# Autodesk Inventor assembly: 00A-200 2019 GreyT Claw
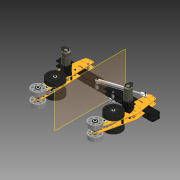
[picture p0: Inventor's stored thumbnail of the model, 180x180]
Saved by Autodesk Inventor 2022 (Build 260153000, 153)
## iProperties
RuleStatus: InUse
Created: 2020-10-29
Part Number: 00A-200 2019 GreyT Claw
Document SubType Name: Assembly
## Documents named in this file (44)
- C:\Users\Cal\Desktop\Robotics\Design\Collaborative\Collaborative Parts Library\Standard Order Parts\GreyT Claw Configurations\GreyT Claw.iam
- C:\Users\Cal\Desktop\Robotics\Design\Collaborative\Collaborative Parts Library\Standard Order Parts\GreyT Claw Configurations\GreyT Claw Top V2.ipt
- C:\Users\Cal\Desktop\Robotics\Design\Collaborative\Collaborative Parts Library\Power Transfer\Bearings and Bushings\Bearings\FR8 Hex.ipt
- D:\FIRST\FRC\1369\CollabPartsLib\Power Transfer\Bearings.ipt
- C:\Users\Cal\Desktop\Robotics\Design\Collaborative\Collaborative Parts Library\Hardware\Spacers\Spacers & Standoffs\VexPro 500 Hex Spacer 0.25in.ipt
- D:\FIRST\FRC\1369\CollabPartsLib\Hardware\Spacers & Standoffs.ipt
- C:\Users\Cal\Desktop\Robotics\Design\Collaborative\Collaborative Parts Library\Power Transfer\Sprockets\Sprockets\VexPro 16T 25 Chain 500 Hex Bore Sprocket.ipt
- D:\FIRST\FRC\1369\CollabPartsLib\Power Transfer\Sprockets\VexPro Sprockets.ipt
- C:\Users\Cal\Desktop\Robotics\Design\Collaborative\Collaborative Parts Library\Hardware\Spacers\Spacers & Standoffs\VexPro 500 Hex Spacer 0.0625in.ipt
- C:\Users\Cal\Desktop\Robotics\Design\Collaborative\Collaborative Parts Library\Hardware\Spacers\Spacers & Standoffs\VexPro 500 Hex Spacer 0.125in.ipt
- C:\Users\Cal\Desktop\Robotics\Design\Collaborative\Collaborative Parts Library\Power Transfer\Hubs (Hex and Key)\Compliant Wheel Hub.ipt
- C:\Users\Cal\Desktop\Robotics\Design\Collaborative\Collaborative Parts Library\Hardware\Spacers\Spacers & Standoffs\Aluminum Hex Standoff (No. 10x32 x 1Lg x 0.375OD).ipt
- C:\Users\Cal\Desktop\Robotics\Design\Collaborative\Collaborative Parts Library\Hardware\Spacers\Spacers & Standoffs\Aluminum Unthreaded Spacer (No. 10 x 1Lg x 0.375OD).ipt
- C:\Users\Cal\Desktop\Robotics\Design\Collaborative\Collaborative Parts Library\General Gearboxes\Planetaries\Versaplanetary\VersaPlanetary\775pro, 2 Stages, 1-2in Hex Output.iam
- D:\FIRST\FRC\1369\CollabPartsLib\Motors\Versaplanetary\VersaPlanetary.iam
- C:\Users\Cal\Desktop\Robotics\Design\Collaborative\Collaborative Parts Library\Hardware\Spacers\Spacers & Standoffs\Aluminum Unthreaded Spacer (0.25in x 1Lg x 0.5OD).ipt
- C:\Users\Cal\Desktop\Robotics\Design\Collaborative\Collaborative Parts Library\Hardware\Spacers\Spacers & Standoffs\Aluminum Unthreaded Spacer (0.25in x 0.5Lg x 0.5OD).ipt
- C:\Users\Cal\Desktop\Robotics\Design\Collaborative\Collaborative Parts Library\Hardware\Spacers\Spacers & Standoffs\Aluminum Hex Standoff (No. 10x32 x 0.875Lg x 0.375OD).ipt
- C:\Users\Cal\Desktop\Robotics\Design\Collaborative\Collaborative Parts Library\Hardware\Spacers\Spacers & Standoffs\Aluminum Unthreaded Spacer (0.25in x 0.438Lg x 0.5OD).ipt
- C:\Users\Cal\Desktop\Robotics\Design\Collaborative\Collaborative Parts Library\Pneumatics\Piston Combined Rod End\.25 in Clevis 6498K42.ipt
- D:\FIRST\FRC\1369\CollabPartsLib\Pneumatics\Piston Combined Rod End.ipt
- C:\Users\Cal\Desktop\Robotics\Design\Collaborative\Collaborative Parts Library\Hardware\Spacers\Spacers & Standoffs\Aluminum Unthreaded Spacer (0.25in x 0.25Lg x 0.5OD).ipt
- C:\Users\Cal\Desktop\Robotics\Design\Collaborative\FRC-Training\19A 2869 or 1836 Concept\19A-200 Intake\19A-200-001 Front Shaft.ipt
- C:\Users\Cal\Desktop\Robotics\Design\Collaborative\FRC-Training\19A 2869 or 1836 Concept\19A-200 Intake\19A-200-002 Mid Shaft.ipt
- C:\Users\Cal\Desktop\Robotics\Design\Collaborative\FRC-Training\19A 2869 or 1836 Concept\19A-200 Intake\19A-200-003 Back Shaft.ipt
- C:\Users\Cal\Desktop\Robotics\Design\Collaborative\Collaborative Parts Library\Hardware\Fasteners\Washers\Washer 0.265ID 0.688OD 0.055Thick.ipt
- D:\FIRST\FRC\1369\CollabPartsLib\Hardware\Washers.ipt
- C:\Users\Cal\Desktop\Robotics\Design\Collaborative\Collaborative Parts Library\Hardware\Fasteners\Machine Screws\1(_FS)4-20 UNCx1 Button Head Cap Screw.ipt
- D:\FIRST\FRC\1369\CollabPartsLib\Hardware\Machine Screws.ipt
- C:\Users\Cal\Desktop\Robotics\Design\Collaborative\Collaborative Parts Library\Hardware\Fasteners\Machine Screws\10-32 UNFx0.5 Socket Head Cap Screw.ipt
- C:\Users\Cal\Desktop\Robotics\Design\Collaborative\Collaborative Parts Library\Standard Order Parts\GreyT Claw Configurations\GrayT Claw Front Chain.ipt
- C:\Users\Cal\Desktop\Robotics\Design\Collaborative\Collaborative Parts Library\Standard Order Parts\GreyT Claw Configurations\GrayT Claw Back Chain.ipt
- C:\Users\Cal\Desktop\Robotics\Design\Collaborative\Collaborative Parts Library\Hardware\Fasteners\Machine Screws\10-32 UNFx1.5 Socket Head Cap Screw.ipt
- C:\Users\Cal\Desktop\Robotics\Design\Collaborative\Collaborative Parts Library\Hardware\Nuts and Threaded Blocks\Nuts\10-32 Pan Head Nylon locknut.ipt
- D:\FIRST\FRC\1369\CollabPartsLib\Hardware\Nuts.ipt
- C:\Users\Cal\Desktop\Robotics\Design\Collaborative\Collaborative Parts Library\Hardware\Fasteners\Machine Screws\10-32 UNFx2.5 Socket Head Cap Screw.ipt
- C:\Users\Cal\Desktop\Robotics\Design\Collaborative\Collaborative Parts Library\Hardware\Fasteners\Machine Screws\10-32 UNFx2.25 Socket Head Cap Screw.ipt
- C:\Users\Cal\Desktop\Robotics\Design\Collaborative\Collaborative Parts Library\Hardware\Fasteners\Washers\Washer 0.203ID 0.438OD 0.038Thick.ipt
- C:\Users\Cal\Desktop\Robotics\Design\Collaborative\Collaborative Parts Library\Wheels\Compliant Wheel Generator\4 in Black 0.5 in Hex Compliant Wheel AM.ipt
- C:\Users\Cal\Desktop\Robotics\Design\Collaborative\Collaborative Parts Library\Wheels and Rollers\Wheels\Compliant Wheel Generator.ipt
- C:\Users\Cal\Desktop\Robotics\Design\Collaborative\Collaborative Parts Library\Wheels\Compliant Wheel Generator\3 in 30A 1.125 in Hex Compliant Wheel VEX.ipt
- C:\Users\Cal\Desktop\Robotics\Design\Collaborative\Collaborative Parts Library\Standard Order Parts\GreyT Claw Configurations\GreyT Claw Wide Plate V2.ipt
- C:\Users\Cal\Desktop\Robotics\Design\Collaborative\Collaborative Parts Library\Pneumatics\Air Cylinder Assembly.iam
- C:\Users\Cal\Desktop\Robotics\Design\Collaborative\Collaborative Parts Library\Pneumatics\Air Cylinder Assembly\2.5 in stroke 0.75 in bore DA Piston.iam
## Components (236 placed, 33 different names)
1. GreyT Claw Top V2:1 — Mate:2, Mate:3, Mate:4, Insert:3, Insert:4, Insert:5, Insert:21, Insert:81, Mate:8, Insert:165, Insert:166, Insert:167, Insert:168, Insert:169, Insert:170, Insert:171, Symmetry:2, Mate:41, Insert:270, Mate:54, Mate:57, Mate:58, Insert:301, Insert:303
2. GreyT Claw Top V2:2 — Mate:2, Mate:3, Mate:4, Insert:6, Insert:7, Insert:8, Insert:9, Insert:55, Insert:56, Insert:57, Insert:58, Insert:59, Insert:60, Insert:71, Insert:73, Insert:74, Insert:172, Insert:173, Insert:174, Insert:175, Insert:176, Insert:177, Insert:178, Insert:195, Insert:196, Mate:33
3. GreyT Claw Top V2:3 — Insert:13, Insert:14, Insert:15, Insert:16, Insert:61, Insert:62, Insert:63, Insert:64, Insert:65, Insert:66, Insert:72, Insert:75, Insert:76, Insert:197, Insert:198, Mate:35, Insert:302, Insert:304
4. GreyT Claw Top V2:4 — Insert:10, Insert:11, Insert:12, Insert:27, Insert:82, Mate:9, Mate:34, Symmetry:2, Mate:40, Insert:271
5. FR8 Hex:1 — Insert:3, Insert:26, Insert:45
6. FR8 Hex:2 — Insert:4, Insert:25, Insert:119
7. FR8 Hex:3 — Insert:5, Insert:17, Insert:23
8. FR8 Hex:4 — Insert:6, Insert:53, Insert:69
9. FR8 Hex:5 — Insert:7
10. FR8 Hex:6 — Insert:8, Insert:49
11. FR8 Hex:7 — Insert:9, Insert:115
12. FR8 Hex:8 — Insert:10, Insert:32, Insert:46
13. FR8 Hex:9 — Insert:11, Insert:31, Insert:120
14. FR8 Hex:10 — Insert:12, Insert:18, Insert:29
15. FR8 Hex:11 — Insert:13, Insert:54, Insert:70
16. FR8 Hex:12 — Insert:14
17. FR8 Hex:13 — Insert:15, Insert:50
18. FR8 Hex:14 — Insert:16, Insert:116
19. VexPro 500 Hex Spacer 0.25in:1 — Insert:17, Insert:19
20. VexPro 500 Hex Spacer 0.25in:2 — Insert:18, Insert:20
21. 4 in Black 0.5 in Hex Compliant Wheel AM:1 — Insert:19, Insert:121
22. 4 in Black 0.5 in Hex Compliant Wheel AM:2 — Insert:20, Insert:122
23. 3 in 30A 1.125 in Hex Compliant Wheel VEX:5 — Insert:43, Insert:117
24. 3 in 30A 1.125 in Hex Compliant Wheel VEX:6 — Insert:44, Insert:118
25. VexPro 16T 25 Chain 500 Hex Bore Sprocket:1 — Insert:21, Insert:41, Insert:79, Mate:28
26. VexPro 16T 25 Chain 500 Hex Bore Sprocket:2 — Insert:22, Insert:23, Mate:27, Mate:29
27. VexPro 16T 25 Chain 500 Hex Bore Sprocket:3 — Insert:22, Mate:19
28. VexPro 16T 25 Chain 500 Hex Bore Sprocket:4 — Insert:24, Insert:25, Mate:16, Mate:17
29. VexPro 16T 25 Chain 500 Hex Bore Sprocket:5 — Insert:24, Mate:18, Mate:20
30. VexPro 16T 25 Chain 500 Hex Bore Sprocket:6 — Insert:26, Mate:15
31. VexPro 16T 25 Chain 500 Hex Bore Sprocket:7 — Insert:27, Insert:42, Insert:80, Mate:31
32. VexPro 16T 25 Chain 500 Hex Bore Sprocket:8 — Insert:28, Insert:29, Mate:30, Mate:32
33. VexPro 16T 25 Chain 500 Hex Bore Sprocket:9 — Insert:28, Mate:24
34. VexPro 16T 25 Chain 500 Hex Bore Sprocket:10 — Insert:30, Insert:31, Mate:22
35. VexPro 16T 25 Chain 500 Hex Bore Sprocket:11 — Insert:30, Mate:23, Mate:26
36. VexPro 16T 25 Chain 500 Hex Bore Sprocket:12 — Insert:32, Mate:21, Mate:25
37. VexPro 500 Hex Spacer 0.25in:5 — Insert:39, Insert:41
38. VexPro 500 Hex Spacer 0.125in:6 — Insert:39
39. VexPro 500 Hex Spacer 0.25in:7 — Insert:42
40. VexPro 500 Hex Spacer 0.125in:8
41. Compliant Wheel Hub:1 — Insert:43, Insert:45
42. Compliant Wheel Hub:2 — Insert:44, Insert:46
43. VexPro 500 Hex Spacer 0.25in:9 — Insert:47, Insert:49
44. 4 in Black 0.5 in Hex Compliant Wheel AM:3 — Insert:47
45. VexPro 500 Hex Spacer 0.25in:10 — Insert:48, Insert:50
46. 4 in Black 0.5 in Hex Compliant Wheel AM:4 — Insert:48
47. 3 in 30A 1.125 in Hex Compliant Wheel VEX:7 — Insert:51
48. Compliant Wheel Hub:3 — Insert:51, Insert:53
49. 3 in 30A 1.125 in Hex Compliant Wheel VEX:8 — Insert:52
50. Compliant Wheel Hub:4 — Insert:52, Insert:54
51. Aluminum Hex Standoff (No. 10x32 x 1Lg x 0.375OD):11 — Insert:56
52. Aluminum Hex Standoff (No. 10x32 x 1Lg x 0.375OD):12 — Insert:55
53. Aluminum Hex Standoff (No. 10x32 x 1Lg x 0.375OD):13 — Insert:58
54. Aluminum Hex Standoff (No. 10x32 x 1Lg x 0.375OD):14 — Insert:57
55. Aluminum Hex Standoff (No. 10x32 x 1Lg x 0.375OD):15 — Insert:60
56. Aluminum Hex Standoff (No. 10x32 x 1Lg x 0.375OD):16 — Insert:59
57. Aluminum Hex Standoff (No. 10x32 x 1Lg x 0.375OD):17 — Insert:62
58. Aluminum Hex Standoff (No. 10x32 x 1Lg x 0.375OD):18 — Insert:61
59. Aluminum Hex Standoff (No. 10x32 x 1Lg x 0.375OD):19 — Insert:64
60. Aluminum Hex Standoff (No. 10x32 x 1Lg x 0.375OD):20 — Insert:63
61. Aluminum Hex Standoff (No. 10x32 x 1Lg x 0.375OD):21 — Insert:66
62. Aluminum Hex Standoff (No. 10x32 x 1Lg x 0.375OD):22 — Insert:65
63. VexPro 500 Hex Spacer 0.25in:23
64. VexPro 500 Hex Spacer 0.125in:24 — Insert:69
65. VexPro 500 Hex Spacer 0.25in:25
66. VexPro 500 Hex Spacer 0.125in:26 — Insert:70
67. Aluminum Hex Standoff (No. 10x32 x 1Lg x 0.375OD):27 — Insert:71
68. Aluminum Hex Standoff (No. 10x32 x 1Lg x 0.375OD):28 — Insert:72
69. Aluminum Unthreaded Spacer (No. 10 x 1Lg x 0.375OD):29 — Insert:73
70. Aluminum Unthreaded Spacer (No. 10 x 1Lg x 0.375OD):30 — Insert:74
71. Aluminum Unthreaded Spacer (No. 10 x 1Lg x 0.375OD):31 — Insert:75
72. Aluminum Unthreaded Spacer (No. 10 x 1Lg x 0.375OD):32 — Insert:76
73. VexPro 500 Hex Spacer 0.125in:33 — Insert:77, Insert:79
74. VexPro 500 Hex Spacer 0.0625in:34 — Insert:77
75. VexPro 500 Hex Spacer 0.125in:35 — Insert:80
76. VexPro 500 Hex Spacer 0.0625in:36
77. 775pro, 2 Stages, 1-2in Hex Output:1 [sub-assembly] — Insert:81, Mate:8, Insert:144
78. 775pro, 2 Stages, 1-2in Hex Output:2 [sub-assembly] — Insert:82, Mate:9, Insert:152
79. VexPro 500 Hex Spacer 0.25in:65 — Insert:115
80. VexPro 500 Hex Spacer 0.25in:66 — Insert:116
81. 19A-200-001 Front Shaft:1 — Insert:117, Insert:147, Insert:150
82. 19A-200-001 Front Shaft:2 — Insert:118, Insert:158, Insert:164
83. 19A-200-002 Mid Shaft:1 — Insert:119, Insert:146, Insert:149
84. 19A-200-002 Mid Shaft:2 — Insert:120, Insert:157, Insert:163
85. 19A-200-003 Back Shaft:1 — Insert:121, Insert:145, Insert:148
86. 19A-200-003 Back Shaft:2 — Insert:122, Insert:156, Insert:162
87. Washer 0.265ID 0.688OD 0.055Thick:1 — Insert:137, Insert:144
88. 1(_FS)4-20 UNCx1 Button Head Cap Screw:1 — Insert:137
89. Washer 0.265ID 0.688OD 0.055Thick:2 — Insert:145
90. 1(_FS)4-20 UNCx1 Button Head Cap Screw:2
91. Washer 0.265ID 0.688OD 0.055Thick:3 — Insert:146
92. 1(_FS)4-20 UNCx1 Button Head Cap Screw:3
93. Washer 0.265ID 0.688OD 0.055Thick:4 — Insert:147
94. 1(_FS)4-20 UNCx1 Button Head Cap Screw:4
95. Washer 0.265ID 0.688OD 0.055Thick:5 — Insert:148
96. 1(_FS)4-20 UNCx1 Button Head Cap Screw:5
97. Washer 0.265ID 0.688OD 0.055Thick:6 — Insert:149
98. 1(_FS)4-20 UNCx1 Button Head Cap Screw:6
99. Washer 0.265ID 0.688OD 0.055Thick:7 — Insert:150
100. 1(_FS)4-20 UNCx1 Button Head Cap Screw:7
101. Washer 0.265ID 0.688OD 0.055Thick:8 — Insert:152
102. 1(_FS)4-20 UNCx1 Button Head Cap Screw:8
103. Washer 0.265ID 0.688OD 0.055Thick:9 — Insert:156
104. 1(_FS)4-20 UNCx1 Button Head Cap Screw:9
105. Washer 0.265ID 0.688OD 0.055Thick:10 — Insert:157
106. 1(_FS)4-20 UNCx1 Button Head Cap Screw:10
107. Washer 0.265ID 0.688OD 0.055Thick:11 — Insert:158
108. 1(_FS)4-20 UNCx1 Button Head Cap Screw:11
109. Washer 0.265ID 0.688OD 0.055Thick:12 — Insert:162
110. 1(_FS)4-20 UNCx1 Button Head Cap Screw:12
111. Washer 0.265ID 0.688OD 0.055Thick:13 — Insert:163
112. 1(_FS)4-20 UNCx1 Button Head Cap Screw:13
113. Washer 0.265ID 0.688OD 0.055Thick:14 — Insert:164
114. 1(_FS)4-20 UNCx1 Button Head Cap Screw:14
115. 10-32 UNFx0.5 Socket Head Cap Screw:15 — Insert:165
116. 10-32 UNFx0.5 Socket Head Cap Screw:16 — Insert:166
117. 10-32 UNFx0.5 Socket Head Cap Screw:17 — Insert:167
118. 10-32 UNFx0.5 Socket Head Cap Screw:18 — Insert:168
119. 10-32 UNFx0.5 Socket Head Cap Screw:19 — Insert:169
120. 10-32 UNFx0.5 Socket Head Cap Screw:20 — Insert:170
121. 10-32 UNFx0.5 Socket Head Cap Screw:21 — Insert:171
122. 10-32 UNFx0.5 Socket Head Cap Screw:22 — Insert:172
123. 10-32 UNFx0.5 Socket Head Cap Screw:23 — Insert:173
124. 10-32 UNFx0.5 Socket Head Cap Screw:24 — Insert:174
125. 10-32 UNFx0.5 Socket Head Cap Screw:25 — Insert:175
126. 10-32 UNFx0.5 Socket Head Cap Screw:26 — Insert:176
127. 10-32 UNFx0.5 Socket Head Cap Screw:27 — Insert:177
128. 10-32 UNFx0.5 Socket Head Cap Screw:28 — Insert:178
129. GrayT Claw Front Chain:1 — Mate:15, Mate:16, Mate:17
130. GrayT Claw Front Chain:2 — Mate:18, Mate:19, Mate:20
131. GrayT Claw Front Chain:3 — Mate:21, Mate:22, Mate:25
132. GrayT Claw Front Chain:4 — Mate:23, Mate:24, Mate:26
133. GrayT Claw Back Chain:1 — Mate:27, Mate:28, Mate:29
134. GrayT Claw Back Chain:2 — Mate:30, Mate:31, Mate:32
135. 10-32 UNFx1.5 Socket Head Cap Screw:45 — Insert:195
136. 10-32 UNFx1.5 Socket Head Cap Screw:46 — Insert:196
137. 10-32 UNFx1.5 Socket Head Cap Screw:47 — Insert:197
138. 10-32 UNFx1.5 Socket Head Cap Screw:48 — Insert:198
139. GreyT Claw Wide Plate V2:1 — Flush:1, Flush:2, Flush:3, Flush:4, Mate:34, Mate:36, Mate:37, Insert:282, Insert:283, Mate:60, Mate:61, Mate:64, Symmetry:1, Mate:65
140. GreyT Claw Wide Plate V2:2 — Mate:33, Flush:1, Flush:4, Mate:35, Angle:4, Symmetry:1
141. 2.5 in stroke 0.75 in bore DA Piston:1 [sub-assembly] — Insert:261, Angle:1, Insert:278, Insert:279
142. .25 in Clevis 6498K42:1 — Insert:261, Angle:1, Insert:274, Insert:275
143. Aluminum Hex Standoff (No. 10x32 x 0.875Lg x 0.375OD):81 — Mate:42
144. Washer 0.203ID 0.438OD 0.038Thick:19 — Insert:270
145. 10-32 UNFx0.5 Socket Head Cap Screw:63 — Mate:44
146. Washer 0.203ID 0.438OD 0.038Thick:20
147. 10-32 UNFx0.5 Socket Head Cap Screw:64
148. Aluminum Hex Standoff (No. 10x32 x 0.875Lg x 0.375OD):82 — Mate:42
149. Washer 0.203ID 0.438OD 0.038Thick:21 — Insert:271
150. 10-32 UNFx0.5 Socket Head Cap Screw:65 — Mate:45
151. Washer 0.203ID 0.438OD 0.038Thick:22
152. 10-32 UNFx0.5 Socket Head Cap Screw:66
153. Aluminum Unthreaded Spacer (0.25in x 0.25Lg x 0.5OD):83 — Insert:272, Insert:274, Insert:301, Insert:303
154. Aluminum Unthreaded Spacer (0.25in x 1Lg x 0.5OD):84 — Insert:272, Insert:273
155. 10-32 Pan Head Nylon locknut:1 — Insert:273
156. 10-32 UNFx2.25 Socket Head Cap Screw:67 — Insert:275
157. Aluminum Unthreaded Spacer (0.25in x 0.438Lg x 0.5OD):85 — Insert:276, Insert:278, Mate:60
158. Aluminum Unthreaded Spacer (0.25in x 1Lg x 0.5OD):86 — Insert:276, Insert:277, Mate:64
159. 10-32 Pan Head Nylon locknut:2 — Insert:277
160. 10-32 UNFx2.5 Socket Head Cap Screw:68 — Insert:279, Mate:62
161. 2.5 in stroke 0.75 in bore DA Piston:2 [sub-assembly]
162. .25 in Clevis 6498K42:2
163. Aluminum Unthreaded Spacer (0.25in x 0.5Lg x 0.5OD):94 — Insert:302, Insert:304
164. Aluminum Unthreaded Spacer (0.25in x 1Lg x 0.5OD):91
165. 10-32 Pan Head Nylon locknut:3
166. 10-32 UNFx2.25 Socket Head Cap Screw:75
167. Aluminum Unthreaded Spacer (0.25in x 0.438Lg x 0.5OD):92 — Mate:61
168. Aluminum Unthreaded Spacer (0.25in x 1Lg x 0.5OD):93 — Mate:65
169. 10-32 Pan Head Nylon locknut:4
170. 10-32 UNFx2.5 Socket Head Cap Screw:76 — Mate:63
171. Aluminum Hex Standoff (No. 10x32 x 1Lg x 0.375OD):87 — Insert:283
172. 10-32 UNFx0.5 Socket Head Cap Screw:70
173. 10-32 UNFx0.5 Socket Head Cap Screw:69
174. Aluminum Hex Standoff (No. 10x32 x 1Lg x 0.375OD):80 — Insert:257, Insert:258, Insert:282
175. 10-32 UNFx0.5 Socket Head Cap Screw:62 — Insert:258
176. 10-32 UNFx0.5 Socket Head Cap Screw:61 — Insert:257
177. Aluminum Hex Standoff (No. 10x32 x 1Lg x 0.375OD):95
178. 10-32 UNFx0.5 Socket Head Cap Screw:77
179. 10-32 UNFx0.5 Socket Head Cap Screw:78
180. Aluminum Hex Standoff (No. 10x32 x 1Lg x 0.375OD):96
181. 10-32 UNFx0.5 Socket Head Cap Screw:79
182. 10-32 UNFx0.5 Socket Head Cap Screw:80
183. Aluminum Hex Standoff (No. 10x32 x 1Lg x 0.375OD):99
184. 10-32 UNFx0.5 Socket Head Cap Screw:85
185. 10-32 UNFx0.5 Socket Head Cap Screw:86
186. Aluminum Hex Standoff (No. 10x32 x 1Lg x 0.375OD):100
187. 10-32 UNFx0.5 Socket Head Cap Screw:87
188. 10-32 UNFx0.5 Socket Head Cap Screw:88
189. Aluminum Hex Standoff (No. 10x32 x 1Lg x 0.375OD):101
190. 10-32 UNFx0.5 Socket Head Cap Screw:89
191. 10-32 UNFx0.5 Socket Head Cap Screw:90
192. Aluminum Hex Standoff (No. 10x32 x 1Lg x 0.375OD):102
193. 10-32 UNFx0.5 Socket Head Cap Screw:91
194. 10-32 UNFx0.5 Socket Head Cap Screw:92
195. Aluminum Hex Standoff (No. 10x32 x 1Lg x 0.375OD):103
196. 10-32 UNFx0.5 Socket Head Cap Screw:93
197. 10-32 UNFx0.5 Socket Head Cap Screw:94
198. Aluminum Hex Standoff (No. 10x32 x 1Lg x 0.375OD):104
199. 10-32 UNFx0.5 Socket Head Cap Screw:95
200. 10-32 UNFx0.5 Socket Head Cap Screw:96
201. Aluminum Hex Standoff (No. 10x32 x 1Lg x 0.375OD):105
202. 10-32 UNFx0.5 Socket Head Cap Screw:97
203. 10-32 UNFx0.5 Socket Head Cap Screw:98
204. Aluminum Hex Standoff (No. 10x32 x 1Lg x 0.375OD):106
205. 10-32 UNFx0.5 Socket Head Cap Screw:99
206. 10-32 UNFx0.5 Socket Head Cap Screw:100
207. Aluminum Hex Standoff (No. 10x32 x 1Lg x 0.375OD):107
208. 10-32 UNFx0.5 Socket Head Cap Screw:101
209. 10-32 UNFx0.5 Socket Head Cap Screw:102
210. Aluminum Hex Standoff (No. 10x32 x 1Lg x 0.375OD):108
211. 10-32 UNFx0.5 Socket Head Cap Screw:103
212. 10-32 UNFx0.5 Socket Head Cap Screw:104
213. Aluminum Hex Standoff (No. 10x32 x 1Lg x 0.375OD):109
214. 10-32 UNFx0.5 Socket Head Cap Screw:105
215. 10-32 UNFx0.5 Socket Head Cap Screw:106
216. Aluminum Hex Standoff (No. 10x32 x 1Lg x 0.375OD):110
217. 10-32 UNFx0.5 Socket Head Cap Screw:107
218. 10-32 UNFx0.5 Socket Head Cap Screw:108
219. Aluminum Hex Standoff (No. 10x32 x 1Lg x 0.375OD):111
220. 10-32 UNFx0.5 Socket Head Cap Screw:109
221. 10-32 UNFx0.5 Socket Head Cap Screw:110
222. Aluminum Hex Standoff (No. 10x32 x 1Lg x 0.375OD):112
223. 10-32 UNFx0.5 Socket Head Cap Screw:111
224. 10-32 UNFx0.5 Socket Head Cap Screw:112
225. Aluminum Hex Standoff (No. 10x32 x 1Lg x 0.375OD):115
226. 10-32 UNFx0.5 Socket Head Cap Screw:117
227. 10-32 UNFx0.5 Socket Head Cap Screw:118
228. Aluminum Hex Standoff (No. 10x32 x 1Lg x 0.375OD):116
229. 10-32 UNFx0.5 Socket Head Cap Screw:119
230. 10-32 UNFx0.5 Socket Head Cap Screw:120
231. Aluminum Hex Standoff (No. 10x32 x 1Lg x 0.375OD):117
232. 10-32 UNFx0.5 Socket Head Cap Screw:121
233. 10-32 UNFx0.5 Socket Head Cap Screw:122
234. Aluminum Hex Standoff (No. 10x32 x 1Lg x 0.375OD):118
235. 10-32 UNFx0.5 Socket Head Cap Screw:123
236. 10-32 UNFx0.5 Socket Head Cap Screw:124
## Component patterns: (13 elements, first: Aluminum Hex Standoff (No. 10x32 x 1Lg x 0.375OD):87 + 10-32 UNFx0.5 Socket Head Cap Screw:70 + 10-32 UNFx0.5 Socket Head Cap Screw:69 + Aluminum Hex Standoff (No. 10x32 x 1Lg x 0.375OD):80 + 10-32 UNFx0.5 Socket Head Cap Screw:62 + 10-32 UNFx0.5 Socket Head Cap Screw:61)
## Relationships (230: Insert 166, Mate 53, Angle 5, Flush 4, Symmetry 2)
- Mate:2: GreyT Claw Top V2:1 ↔ GreyT Claw Top V2:2
- Mate:3: GreyT Claw Top V2:1 ↔ GreyT Claw Top V2:2
- Mate:4 (25.4 mm): GreyT Claw Top V2:1 ↔ GreyT Claw Top V2:2
- [Mate]: GreyT Claw Top V2:3 ↔ GreyT Claw Top V2:4
- [Mate]: GreyT Claw Top V2:3 ↔ GreyT Claw Top V2:4
- [Mate] (25.4 mm): GreyT Claw Top V2:3 ↔ GreyT Claw Top V2:4
- Insert:3: GreyT Claw Top V2:1 ↔ FR8 Hex:1
- Insert:4: GreyT Claw Top V2:1 ↔ FR8 Hex:2
- Insert:5: GreyT Claw Top V2:1 ↔ FR8 Hex:3
- Insert:6: GreyT Claw Top V2:2 ↔ FR8 Hex:4
- Insert:7: GreyT Claw Top V2:2 ↔ FR8 Hex:5
- Insert:8: GreyT Claw Top V2:2 ↔ FR8 Hex:6
- Insert:9: GreyT Claw Top V2:2 ↔ FR8 Hex:7
- Insert:10: GreyT Claw Top V2:4 ↔ FR8 Hex:8
- Insert:11: GreyT Claw Top V2:4 ↔ FR8 Hex:9
- Insert:12: GreyT Claw Top V2:4 ↔ FR8 Hex:10
- Insert:13: GreyT Claw Top V2:3 ↔ FR8 Hex:11
- Insert:14: GreyT Claw Top V2:3 ↔ FR8 Hex:12
- Insert:15: GreyT Claw Top V2:3 ↔ FR8 Hex:13
- Insert:16: GreyT Claw Top V2:3 ↔ FR8 Hex:14
- Insert:17: FR8 Hex:3 ↔ VexPro 500 Hex Spacer 0.25in:1
- Insert:18: FR8 Hex:10 ↔ VexPro 500 Hex Spacer 0.25in:2
- Insert:19: VexPro 500 Hex Spacer 0.25in:1 ↔ 4 in Black 0.5 in Hex Compliant Wheel AM:1
- Insert:20: VexPro 500 Hex Spacer 0.25in:2 ↔ 4 in Black 0.5 in Hex Compliant Wheel AM:2
- Insert:21 (3.175 mm): GreyT Claw Top V2:1 ↔ VexPro 16T 25 Chain 500 Hex Bore Sprocket:1
- Insert:22: VexPro 16T 25 Chain 500 Hex Bore Sprocket:2 ↔ VexPro 16T 25 Chain 500 Hex Bore Sprocket:3
- Insert:23: FR8 Hex:3 ↔ VexPro 16T 25 Chain 500 Hex Bore Sprocket:2
- Insert:24: VexPro 16T 25 Chain 500 Hex Bore Sprocket:4 ↔ VexPro 16T 25 Chain 500 Hex Bore Sprocket:5
- Insert:25: FR8 Hex:2 ↔ VexPro 16T 25 Chain 500 Hex Bore Sprocket:4
- Insert:26: FR8 Hex:1 ↔ VexPro 16T 25 Chain 500 Hex Bore Sprocket:6
- Insert:27 (3.175 mm): GreyT Claw Top V2:4 ↔ VexPro 16T 25 Chain 500 Hex Bore Sprocket:7
- Insert:28: VexPro 16T 25 Chain 500 Hex Bore Sprocket:8 ↔ VexPro 16T 25 Chain 500 Hex Bore Sprocket:9
- Insert:29: FR8 Hex:10 ↔ VexPro 16T 25 Chain 500 Hex Bore Sprocket:8
- Insert:30: VexPro 16T 25 Chain 500 Hex Bore Sprocket:10 ↔ VexPro 16T 25 Chain 500 Hex Bore Sprocket:11
- Insert:31: FR8 Hex:9 ↔ VexPro 16T 25 Chain 500 Hex Bore Sprocket:10
- Insert:32: FR8 Hex:8 ↔ VexPro 16T 25 Chain 500 Hex Bore Sprocket:12
- Insert:39: VexPro 500 Hex Spacer 0.25in:5 ↔ VexPro 500 Hex Spacer 0.125in:6
- [Insert]: VexPro 500 Hex Spacer 0.25in:7 ↔ VexPro 500 Hex Spacer 0.125in:8
- Insert:41: VexPro 16T 25 Chain 500 Hex Bore Sprocket:1 ↔ VexPro 500 Hex Spacer 0.25in:5
- Insert:42: VexPro 16T 25 Chain 500 Hex Bore Sprocket:7 ↔ VexPro 500 Hex Spacer 0.25in:7
- Insert:43: 3 in 30A 1.125 in Hex Compliant Wheel VEX:5 ↔ Compliant Wheel Hub:1
- Insert:44: 3 in 30A 1.125 in Hex Compliant Wheel VEX:6 ↔ Compliant Wheel Hub:2
- Insert:45: FR8 Hex:1 ↔ Compliant Wheel Hub:1
- Insert:46: FR8 Hex:8 ↔ Compliant Wheel Hub:2
- Insert:47: VexPro 500 Hex Spacer 0.25in:9 ↔ 4 in Black 0.5 in Hex Compliant Wheel AM:3
- Insert:48: VexPro 500 Hex Spacer 0.25in:10 ↔ 4 in Black 0.5 in Hex Compliant Wheel AM:4
- Insert:49: FR8 Hex:6 ↔ VexPro 500 Hex Spacer 0.25in:9
- Insert:50: FR8 Hex:13 ↔ VexPro 500 Hex Spacer 0.25in:10
- Insert:51: 3 in 30A 1.125 in Hex Compliant Wheel VEX:7 ↔ Compliant Wheel Hub:3
- Insert:52: 3 in 30A 1.125 in Hex Compliant Wheel VEX:8 ↔ Compliant Wheel Hub:4
- Insert:53: FR8 Hex:4 ↔ Compliant Wheel Hub:3
- Insert:54: FR8 Hex:11 ↔ Compliant Wheel Hub:4
- Insert:55: GreyT Claw Top V2:2 ↔ Aluminum Hex Standoff (No. 10x32 x 1Lg x 0.375OD):12
- Insert:56: GreyT Claw Top V2:2 ↔ Aluminum Hex Standoff (No. 10x32 x 1Lg x 0.375OD):11
- Insert:57: GreyT Claw Top V2:2 ↔ Aluminum Hex Standoff (No. 10x32 x 1Lg x 0.375OD):14
- Insert:58: GreyT Claw Top V2:2 ↔ Aluminum Hex Standoff (No. 10x32 x 1Lg x 0.375OD):13
- Insert:59: GreyT Claw Top V2:2 ↔ Aluminum Hex Standoff (No. 10x32 x 1Lg x 0.375OD):16
- Insert:60: GreyT Claw Top V2:2 ↔ Aluminum Hex Standoff (No. 10x32 x 1Lg x 0.375OD):15
- Insert:61: GreyT Claw Top V2:3 ↔ Aluminum Hex Standoff (No. 10x32 x 1Lg x 0.375OD):18
- Insert:62: GreyT Claw Top V2:3 ↔ Aluminum Hex Standoff (No. 10x32 x 1Lg x 0.375OD):17
- Insert:63: GreyT Claw Top V2:3 ↔ Aluminum Hex Standoff (No. 10x32 x 1Lg x 0.375OD):20
- Insert:64: GreyT Claw Top V2:3 ↔ Aluminum Hex Standoff (No. 10x32 x 1Lg x 0.375OD):19
- Insert:65: GreyT Claw Top V2:3 ↔ Aluminum Hex Standoff (No. 10x32 x 1Lg x 0.375OD):22
- Insert:66: GreyT Claw Top V2:3 ↔ Aluminum Hex Standoff (No. 10x32 x 1Lg x 0.375OD):21
- [Insert]: VexPro 500 Hex Spacer 0.25in:23 ↔ VexPro 500 Hex Spacer 0.125in:24
- [Insert]: VexPro 500 Hex Spacer 0.25in:25 ↔ VexPro 500 Hex Spacer 0.125in:26
- Insert:69: FR8 Hex:4 ↔ VexPro 500 Hex Spacer 0.125in:24
- Insert:70: FR8 Hex:11 ↔ VexPro 500 Hex Spacer 0.125in:26
- Insert:71: GreyT Claw Top V2:2 ↔ Aluminum Hex Standoff (No. 10x32 x 1Lg x 0.375OD):27
- Insert:72: GreyT Claw Top V2:3 ↔ Aluminum Hex Standoff (No. 10x32 x 1Lg x 0.375OD):28
- Insert:73: GreyT Claw Top V2:2 ↔ Aluminum Unthreaded Spacer (No. 10 x 1Lg x 0.375OD):29
- Insert:74: GreyT Claw Top V2:2 ↔ Aluminum Unthreaded Spacer (No. 10 x 1Lg x 0.375OD):30
- Insert:75: GreyT Claw Top V2:3 ↔ Aluminum Unthreaded Spacer (No. 10 x 1Lg x 0.375OD):31
- Insert:76: GreyT Claw Top V2:3 ↔ Aluminum Unthreaded Spacer (No. 10 x 1Lg x 0.375OD):32
- Insert:77: VexPro 500 Hex Spacer 0.125in:33 ↔ VexPro 500 Hex Spacer 0.0625in:34
- [Insert]: VexPro 500 Hex Spacer 0.125in:35 ↔ VexPro 500 Hex Spacer 0.0625in:36
- Insert:79: VexPro 16T 25 Chain 500 Hex Bore Sprocket:1 ↔ VexPro 500 Hex Spacer 0.125in:33
- Insert:80: VexPro 16T 25 Chain 500 Hex Bore Sprocket:7 ↔ VexPro 500 Hex Spacer 0.125in:35
- Insert:81: GreyT Claw Top V2:1 ↔ 775pro, 2 Stages, 1-2in Hex Output:1
- Insert:82: GreyT Claw Top V2:4 ↔ 775pro, 2 Stages, 1-2in Hex Output:2
- Mate:8: GreyT Claw Top V2:1 ↔ 775pro, 2 Stages, 1-2in Hex Output:1
- Mate:9: GreyT Claw Top V2:4 ↔ 775pro, 2 Stages, 1-2in Hex Output:2
- Insert:115: FR8 Hex:7 ↔ VexPro 500 Hex Spacer 0.25in:65
- Insert:116: FR8 Hex:14 ↔ VexPro 500 Hex Spacer 0.25in:66
- Insert:117: 3 in 30A 1.125 in Hex Compliant Wheel VEX:5 ↔ 19A-200-001 Front Shaft:1
- Insert:118: 3 in 30A 1.125 in Hex Compliant Wheel VEX:6 ↔ 19A-200-001 Front Shaft:2
- Insert:119: FR8 Hex:2 ↔ 19A-200-002 Mid Shaft:1
- Insert:120: FR8 Hex:9 ↔ 19A-200-002 Mid Shaft:2
- Insert:121: 4 in Black 0.5 in Hex Compliant Wheel AM:1 ↔ 19A-200-003 Back Shaft:1
- Insert:122: 4 in Black 0.5 in Hex Compliant Wheel AM:2 ↔ 19A-200-003 Back Shaft:2
- Insert:137: Washer 0.265ID 0.688OD 0.055Thick:1 ↔ 1(_FS)4-20 UNCx1 Button Head Cap Screw:1
- [Insert]: Washer 0.265ID 0.688OD 0.055Thick:2 ↔ 1(_FS)4-20 UNCx1 Button Head Cap Screw:2
- [Insert]: Washer 0.265ID 0.688OD 0.055Thick:3 ↔ 1(_FS)4-20 UNCx1 Button Head Cap Screw:3
- [Insert]: Washer 0.265ID 0.688OD 0.055Thick:4 ↔ 1(_FS)4-20 UNCx1 Button Head Cap Screw:4
- [Insert]: Washer 0.265ID 0.688OD 0.055Thick:5 ↔ 1(_FS)4-20 UNCx1 Button Head Cap Screw:5
- [Insert]: Washer 0.265ID 0.688OD 0.055Thick:6 ↔ 1(_FS)4-20 UNCx1 Button Head Cap Screw:6
- [Insert]: Washer 0.265ID 0.688OD 0.055Thick:7 ↔ 1(_FS)4-20 UNCx1 Button Head Cap Screw:7
- Insert:144: 775pro, 2 Stages, 1-2in Hex Output:1 ↔ Washer 0.265ID 0.688OD 0.055Thick:1
- Insert:145: 19A-200-003 Back Shaft:1 ↔ Washer 0.265ID 0.688OD 0.055Thick:2
- Insert:146: 19A-200-002 Mid Shaft:1 ↔ Washer 0.265ID 0.688OD 0.055Thick:3
- Insert:147: 19A-200-001 Front Shaft:1 ↔ Washer 0.265ID 0.688OD 0.055Thick:4
- Insert:148: 19A-200-003 Back Shaft:1 ↔ Washer 0.265ID 0.688OD 0.055Thick:5
- Insert:149: 19A-200-002 Mid Shaft:1 ↔ Washer 0.265ID 0.688OD 0.055Thick:6
- Insert:150: 19A-200-001 Front Shaft:1 ↔ Washer 0.265ID 0.688OD 0.055Thick:7
- [Insert]: Washer 0.265ID 0.688OD 0.055Thick:8 ↔ 1(_FS)4-20 UNCx1 Button Head Cap Screw:8
- Insert:152: 775pro, 2 Stages, 1-2in Hex Output:2 ↔ Washer 0.265ID 0.688OD 0.055Thick:8
- [Insert]: Washer 0.265ID 0.688OD 0.055Thick:9 ↔ 1(_FS)4-20 UNCx1 Button Head Cap Screw:9
- [Insert]: Washer 0.265ID 0.688OD 0.055Thick:10 ↔ 1(_FS)4-20 UNCx1 Button Head Cap Screw:10
- [Insert]: Washer 0.265ID 0.688OD 0.055Thick:11 ↔ 1(_FS)4-20 UNCx1 Button Head Cap Screw:11
- Insert:156: 19A-200-003 Back Shaft:2 ↔ Washer 0.265ID 0.688OD 0.055Thick:9
- Insert:157: 19A-200-002 Mid Shaft:2 ↔ Washer 0.265ID 0.688OD 0.055Thick:10
- Insert:158: 19A-200-001 Front Shaft:2 ↔ Washer 0.265ID 0.688OD 0.055Thick:11
- [Insert]: Washer 0.265ID 0.688OD 0.055Thick:12 ↔ 1(_FS)4-20 UNCx1 Button Head Cap Screw:12
- [Insert]: Washer 0.265ID 0.688OD 0.055Thick:13 ↔ 1(_FS)4-20 UNCx1 Button Head Cap Screw:13
- [Insert]: Washer 0.265ID 0.688OD 0.055Thick:14 ↔ 1(_FS)4-20 UNCx1 Button Head Cap Screw:14
- Insert:162: 19A-200-003 Back Shaft:2 ↔ Washer 0.265ID 0.688OD 0.055Thick:12
- Insert:163: 19A-200-002 Mid Shaft:2 ↔ Washer 0.265ID 0.688OD 0.055Thick:13
- Insert:164: 19A-200-001 Front Shaft:2 ↔ Washer 0.265ID 0.688OD 0.055Thick:14
- Insert:165: GreyT Claw Top V2:1 ↔ 10-32 UNFx0.5 Socket Head Cap Screw:15
- Insert:166: GreyT Claw Top V2:1 ↔ 10-32 UNFx0.5 Socket Head Cap Screw:16
- Insert:167: GreyT Claw Top V2:1 ↔ 10-32 UNFx0.5 Socket Head Cap Screw:17
- Insert:168: GreyT Claw Top V2:1 ↔ 10-32 UNFx0.5 Socket Head Cap Screw:18
- Insert:169: GreyT Claw Top V2:1 ↔ 10-32 UNFx0.5 Socket Head Cap Screw:19
- Insert:170: GreyT Claw Top V2:1 ↔ 10-32 UNFx0.5 Socket Head Cap Screw:20
- Insert:171: GreyT Claw Top V2:1 ↔ 10-32 UNFx0.5 Socket Head Cap Screw:21
- Insert:172: GreyT Claw Top V2:2 ↔ 10-32 UNFx0.5 Socket Head Cap Screw:22
- Insert:173: GreyT Claw Top V2:2 ↔ 10-32 UNFx0.5 Socket Head Cap Screw:23
- Insert:174: GreyT Claw Top V2:2 ↔ 10-32 UNFx0.5 Socket Head Cap Screw:24
- Insert:175: GreyT Claw Top V2:2 ↔ 10-32 UNFx0.5 Socket Head Cap Screw:25
- Insert:176: GreyT Claw Top V2:2 ↔ 10-32 UNFx0.5 Socket Head Cap Screw:26
- Insert:177: GreyT Claw Top V2:2 ↔ 10-32 UNFx0.5 Socket Head Cap Screw:27
- Insert:178: GreyT Claw Top V2:2 ↔ 10-32 UNFx0.5 Socket Head Cap Screw:28
- Mate:15: VexPro 16T 25 Chain 500 Hex Bore Sprocket:6 ↔ GrayT Claw Front Chain:1
- Mate:16: VexPro 16T 25 Chain 500 Hex Bore Sprocket:4 ↔ GrayT Claw Front Chain:1
- Mate:17: VexPro 16T 25 Chain 500 Hex Bore Sprocket:4 ↔ GrayT Claw Front Chain:1
- Mate:18: VexPro 16T 25 Chain 500 Hex Bore Sprocket:5 ↔ GrayT Claw Front Chain:2
- Mate:19: VexPro 16T 25 Chain 500 Hex Bore Sprocket:3 ↔ GrayT Claw Front Chain:2
- Mate:20: VexPro 16T 25 Chain 500 Hex Bore Sprocket:5 ↔ GrayT Claw Front Chain:2
- Mate:21: VexPro 16T 25 Chain 500 Hex Bore Sprocket:12 ↔ GrayT Claw Front Chain:3
- Mate:22: VexPro 16T 25 Chain 500 Hex Bore Sprocket:10 ↔ GrayT Claw Front Chain:3
- Mate:23: VexPro 16T 25 Chain 500 Hex Bore Sprocket:11 ↔ GrayT Claw Front Chain:4
- Mate:24: VexPro 16T 25 Chain 500 Hex Bore Sprocket:9 ↔ GrayT Claw Front Chain:4
- Mate:25: VexPro 16T 25 Chain 500 Hex Bore Sprocket:12 ↔ GrayT Claw Front Chain:3
- Mate:26: VexPro 16T 25 Chain 500 Hex Bore Sprocket:11 ↔ GrayT Claw Front Chain:4
- Mate:27: VexPro 16T 25 Chain 500 Hex Bore Sprocket:2 ↔ GrayT Claw Back Chain:1
- Mate:28: VexPro 16T 25 Chain 500 Hex Bore Sprocket:1 ↔ GrayT Claw Back Chain:1
- Mate:29: VexPro 16T 25 Chain 500 Hex Bore Sprocket:2 ↔ GrayT Claw Back Chain:1
- Mate:30: VexPro 16T 25 Chain 500 Hex Bore Sprocket:8 ↔ GrayT Claw Back Chain:2
- Mate:31: VexPro 16T 25 Chain 500 Hex Bore Sprocket:7 ↔ GrayT Claw Back Chain:2
- Mate:32: VexPro 16T 25 Chain 500 Hex Bore Sprocket:8 ↔ GrayT Claw Back Chain:2
- Insert:195: GreyT Claw Top V2:2 ↔ 10-32 UNFx1.5 Socket Head Cap Screw:45
- Insert:196: GreyT Claw Top V2:2 ↔ 10-32 UNFx1.5 Socket Head Cap Screw:46
- Insert:197: GreyT Claw Top V2:3 ↔ 10-32 UNFx1.5 Socket Head Cap Screw:47
- Insert:198: GreyT Claw Top V2:3 ↔ 10-32 UNFx1.5 Socket Head Cap Screw:48
- Insert:257 (3.175 mm): Aluminum Hex Standoff (No. 10x32 x 1Lg x 0.375OD):80 ↔ 10-32 UNFx0.5 Socket Head Cap Screw:61
- Insert:258 (3.175 mm): Aluminum Hex Standoff (No. 10x32 x 1Lg x 0.375OD):80 ↔ 10-32 UNFx0.5 Socket Head Cap Screw:62
- Mate:33: GreyT Claw Top V2:2 ↔ GreyT Claw Wide Plate V2:2
- Flush:1: GreyT Claw Wide Plate V2:1 ↔ GreyT Claw Wide Plate V2:2
- Flush:2: GreyT Claw Wide Plate V2:1
- Flush:3: GreyT Claw Wide Plate V2:1
- Flush:4: GreyT Claw Wide Plate V2:1 ↔ GreyT Claw Wide Plate V2:2
- Symmetry:1: GreyT Claw Wide Plate V2:1 ↔ GreyT Claw Wide Plate V2:2
- Mate:34: GreyT Claw Top V2:4 ↔ GreyT Claw Wide Plate V2:1
- Symmetry:2: GreyT Claw Top V2:1 ↔ GreyT Claw Top V2:4
- Mate:35: GreyT Claw Top V2:3 ↔ GreyT Claw Wide Plate V2:2
- Mate:36: GreyT Claw Wide Plate V2:1
- Mate:37: GreyT Claw Wide Plate V2:1
- Mate:38
- Mate:39
- Mate:40: GreyT Claw Top V2:4
- Mate:41: GreyT Claw Top V2:1
- Insert:261: 2.5 in stroke 0.75 in bore DA Piston:1 ↔ .25 in Clevis 6498K42:1
- Angle:1 (0 deg): 2.5 in stroke 0.75 in bore DA Piston:1 ↔ .25 in Clevis 6498K42:1
- [Insert]: Washer 0.203ID 0.438OD 0.038Thick:19 ↔ 10-32 UNFx0.5 Socket Head Cap Screw:63
- [Insert]: Washer 0.203ID 0.438OD 0.038Thick:20 ↔ 10-32 UNFx0.5 Socket Head Cap Screw:64
- [Insert] (6.35 mm): Aluminum Hex Standoff (No. 10x32 x 0.875Lg x 0.375OD):81 ↔ Washer 0.203ID 0.438OD 0.038Thick:19
- [Insert] (6.35 mm): Aluminum Hex Standoff (No. 10x32 x 0.875Lg x 0.375OD):81 ↔ Washer 0.203ID 0.438OD 0.038Thick:20
- [Insert]: Washer 0.203ID 0.438OD 0.038Thick:21 ↔ 10-32 UNFx0.5 Socket Head Cap Screw:65
- [Insert]: Washer 0.203ID 0.438OD 0.038Thick:22 ↔ 10-32 UNFx0.5 Socket Head Cap Screw:66
- [Insert] (6.35 mm): Aluminum Hex Standoff (No. 10x32 x 0.875Lg x 0.375OD):82 ↔ Washer 0.203ID 0.438OD 0.038Thick:21
- [Insert] (6.35 mm): Aluminum Hex Standoff (No. 10x32 x 0.875Lg x 0.375OD):82 ↔ Washer 0.203ID 0.438OD 0.038Thick:22
- Insert:270: GreyT Claw Top V2:1 ↔ Washer 0.203ID 0.438OD 0.038Thick:19
- Insert:271: GreyT Claw Top V2:4 ↔ Washer 0.203ID 0.438OD 0.038Thick:21
- Insert:272 (3.175 mm): Aluminum Unthreaded Spacer (0.25in x 0.25Lg x 0.5OD):83 ↔ Aluminum Unthreaded Spacer (0.25in x 1Lg x 0.5OD):84
- Insert:273 (3.175 mm): Aluminum Unthreaded Spacer (0.25in x 1Lg x 0.5OD):84 ↔ 10-32 Pan Head Nylon locknut:1
- Insert:274: .25 in Clevis 6498K42:1 ↔ Aluminum Unthreaded Spacer (0.25in x 0.25Lg x 0.5OD):83
- Insert:275: .25 in Clevis 6498K42:1 ↔ 10-32 UNFx2.25 Socket Head Cap Screw:67
- Insert:276 (3.175 mm): Aluminum Unthreaded Spacer (0.25in x 0.438Lg x 0.5OD):85 ↔ Aluminum Unthreaded Spacer (0.25in x 1Lg x 0.5OD):86
- Insert:277 (3.175 mm): Aluminum Unthreaded Spacer (0.25in x 1Lg x 0.5OD):86 ↔ 10-32 Pan Head Nylon locknut:2
- Insert:278: 2.5 in stroke 0.75 in bore DA Piston:1 ↔ Aluminum Unthreaded Spacer (0.25in x 0.438Lg x 0.5OD):85
- Insert:279: 2.5 in stroke 0.75 in bore DA Piston:1 ↔ 10-32 UNFx2.5 Socket Head Cap Screw:68
- Mate:42 (381 mm): Aluminum Hex Standoff (No. 10x32 x 0.875Lg x 0.375OD):81 ↔ Aluminum Hex Standoff (No. 10x32 x 0.875Lg x 0.375OD):82
- [Insert] (3.175 mm): Aluminum Hex Standoff (No. 10x32 x 1Lg x 0.375OD):87 ↔ 10-32 UNFx0.5 Socket Head Cap Screw:69
- [Insert] (3.175 mm): Aluminum Hex Standoff (No. 10x32 x 1Lg x 0.375OD):87 ↔ 10-32 UNFx0.5 Socket Head Cap Screw:70
- Insert:282: GreyT Claw Wide Plate V2:1 ↔ Aluminum Hex Standoff (No. 10x32 x 1Lg x 0.375OD):80
- Insert:283: GreyT Claw Wide Plate V2:1 ↔ Aluminum Hex Standoff (No. 10x32 x 1Lg x 0.375OD):87
- Mate:44: 10-32 UNFx0.5 Socket Head Cap Screw:63
- Mate:45: 10-32 UNFx0.5 Socket Head Cap Screw:65
- Mate:47
- Mate:48
- Mate:49
- Mate:50
- Mate:51
- Mate:52
- Angle:3 (0 deg)
- Angle:4 (0 deg): GreyT Claw Wide Plate V2:2
- Angle:5 (90 deg)
- Mate:54: GreyT Claw Top V2:1
- Mate:57: GreyT Claw Top V2:1
- Mate:58: GreyT Claw Top V2:1
- [Insert]: 2.5 in stroke 0.75 in bore DA Piston:2 ↔ .25 in Clevis 6498K42:2
- [Angle] (0 deg): 2.5 in stroke 0.75 in bore DA Piston:2 ↔ .25 in Clevis 6498K42:2
- [Insert] (3.175 mm): Aluminum Unthreaded Spacer (0.25in x 0.5Lg x 0.5OD):94 ↔ Aluminum Unthreaded Spacer (0.25in x 1Lg x 0.5OD):91
- [Insert] (3.175 mm): Aluminum Unthreaded Spacer (0.25in x 1Lg x 0.5OD):91 ↔ 10-32 Pan Head Nylon locknut:3
- [Insert]: .25 in Clevis 6498K42:2 ↔ Aluminum Unthreaded Spacer (0.25in x 0.5Lg x 0.5OD):94
- [Insert]: .25 in Clevis 6498K42:2 ↔ 10-32 UNFx2.25 Socket Head Cap Screw:75
- [Insert] (3.175 mm): Aluminum Unthreaded Spacer (0.25in x 0.438Lg x 0.5OD):92 ↔ Aluminum Unthreaded Spacer (0.25in x 1Lg x 0.5OD):93
- [Insert] (3.175 mm): Aluminum Unthreaded Spacer (0.25in x 1Lg x 0.5OD):93 ↔ 10-32 Pan Head Nylon locknut:4
- [Insert]: 2.5 in stroke 0.75 in bore DA Piston:2 ↔ Aluminum Unthreaded Spacer (0.25in x 0.438Lg x 0.5OD):92
- [Insert]: 2.5 in stroke 0.75 in bore DA Piston:2 ↔ 10-32 UNFx2.5 Socket Head Cap Screw:76
- Insert:301: GreyT Claw Top V2:1 ↔ Aluminum Unthreaded Spacer (0.25in x 0.25Lg x 0.5OD):83
- Mate:60 (-6.35 mm): GreyT Claw Wide Plate V2:1 ↔ Aluminum Unthreaded Spacer (0.25in x 0.438Lg x 0.5OD):85
- Insert:302: GreyT Claw Top V2:3 ↔ Aluminum Unthreaded Spacer (0.25in x 0.5Lg x 0.5OD):94
- Mate:61 (-6.35 mm): GreyT Claw Wide Plate V2:1 ↔ Aluminum Unthreaded Spacer (0.25in x 0.438Lg x 0.5OD):92
- Mate:62: 10-32 UNFx2.5 Socket Head Cap Screw:68
- Mate:63: 10-32 UNFx2.5 Socket Head Cap Screw:76
- Mate:64 (-260.35 mm): GreyT Claw Wide Plate V2:1 ↔ Aluminum Unthreaded Spacer (0.25in x 1Lg x 0.5OD):86
- Mate:65 (-260.35 mm): GreyT Claw Wide Plate V2:1 ↔ Aluminum Unthreaded Spacer (0.25in x 1Lg x 0.5OD):93
- Insert:303: GreyT Claw Top V2:1 ↔ Aluminum Unthreaded Spacer (0.25in x 0.25Lg x 0.5OD):83
- Insert:304: GreyT Claw Top V2:3 ↔ Aluminum Unthreaded Spacer (0.25in x 0.5Lg x 0.5OD):94
## Named parameters: d7_d3 = 0 mm, d8_d4 = 0 mm, d9_d5 = 25.4 mm, d50_d49 = 0 mm, d57_d27 = 0 mm, d58_d27 = 0 mm, d61_d53 = 0 mm, d62_d53 = 0 mm, d77_d49 = 0 mm, d78_d49 = 0 mm, d88_d87 = 0 mm, d169_d168 = 0 mm, d170_d168 = 0 mm, d171_d168 = 0 mm, d172_d168 = 0 mm, d173_d168 = 0 mm, d174_d168 = 0 mm, d182_d168 = 0 mm, d184_d168 = 0 mm, d185_d168 = 0 mm, d186_d168 = 0 mm, d190_d168 = 0 mm, d191_d168 = 0 mm, d192_d168 = 0 mm, d349_d337 = 6.35 mm, d350_d338 = 6.35 mm, d351_d259 = 0 mm, d352_d264_d259 = 0 mm, d353_d349_d337 = 6.35 mm, d354_d350_d338 = 6.35 mm, d355_d351_d259 = 0 mm, d356_d352_d264_d259 = 0 mm, Pivot_Distance = 381 mm, d368_d330 = 3.175 mm, d369_d331 = 3.175 mm, d412_d364 = 3.175 mm, d413_d365 = 0 mm, d414_d366 = 0 mm, d415_d347 = 0 mm, d416_d348 = 0 deg, d417_d359 = 3.175 mm, d418_d360 = 3.175 mm, d419_d361 = 0 mm, d420_d362 = 0 mm, d421_d363 = 3.175 mm, Pneumatic_Spacing = -260.35 mm
